# Autodesk Inventor assembly: v2RevA
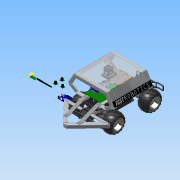
[picture p0: Inventor's stored thumbnail of the model, 180x180]
Saved by Autodesk Inventor 2014 (Build 180170000, 170)
## iProperties
Created: 2013-12-30
Part Number: v2RevA
Document SubType Name: Assembly
Designer: davidgitz
Author: davidgitz
## Documents named in this file (40)
- C:\SharedDrive\Dropbox\ICARUS\Rover\v2-Mechanical\v2RevA.iam
- C:\SharedDrive\Dropbox\ICARUS\Rover\v2-Mechanical\Frame\FrameMember.ipt
- C:\SharedDrive\Dropbox\ICARUS\Rover\v2-Mechanical\Frame\Hex Offset.ipt
- C:\SharedDrive\Dropbox\ICARUS\Rover\v2-Mechanical\Frame\Plate.ipt
- C:\SharedDrive\Dropbox\ICARUS\Rover\v2-Mechanical\Electronics\IFI,VICTOR,Victor 884\IFI,VICTOR,Victor 884.iam
- C:\SharedDrive\Dropbox\ICARUS\Rover\v2-Mechanical\Electronics\FuseBlock.ipt
- C:\SharedDrive\Dropbox\ICARUS\Rover\v2-Mechanical\Electronics\Terminal Block.ipt
- C:\SharedDrive\Dropbox\ICARUS\Rover\v2-Mechanical\H2 OEM\Drive Axle.ipt
- C:\SharedDrive\Dropbox\ICARUS\Rover\v2-Mechanical\H2 OEM\Rear Axle Housing.ipt
- C:\SharedDrive\Dropbox\ICARUS\Rover\v2-Mechanical\H2 OEM\Elec Cover.ipt
- C:\SharedDrive\Dropbox\ICARUS\Rover\v2-Mechanical\H2 OEM\Shock Plate - Top (Left).ipt
- C:\SharedDrive\Dropbox\ICARUS\Rover\v2-Mechanical\H2 OEM\Shock Plate - Bottom (Left).ipt
- C:\SharedDrive\Dropbox\ICARUS\Rover\v2-Mechanical\H2 OEM\Shock Plate - Bottom (Right).ipt
- C:\SharedDrive\Dropbox\ICARUS\Rover\v2-Mechanical\H2 OEM\Shock Plate - Top (Right).ipt
- C:\SharedDrive\Dropbox\ICARUS\Rover\v2-Mechanical\H2 OEM\Shock Mount - Top.ipt
- C:\SharedDrive\Dropbox\ICARUS\Rover\v2-Mechanical\Imported Components\Final\Final.iam
- C:\SharedDrive\Dropbox\ICARUS\Rover\v2-Mechanical\Imported Components\ArduinoMega2560R3\ArduinoMega2560R3.iam
- C:\SharedDrive\Dropbox\ICARUS\Rover\v2-Mechanical\Electronics\GBS-20132-EL2.ipt
- C:\SharedDrive\Dropbox\ICARUS\Rover\v2-Mechanical\H2 OEM\FrontHousing.ipt
- C:\SharedDrive\Dropbox\ICARUS\Rover\v2-Mechanical\H2 OEM\RearHousing.ipt
- C:\SharedDrive\Dropbox\ICARUS\Rover\v2-Mechanical\H2 OEM\LargeLeftWheel.ipt
- C:\SharedDrive\Dropbox\ICARUS\Rover\v2-Mechanical\H2 OEM\LargeRightWheel.ipt
- C:\SharedDrive\Dropbox\ICARUS\Rover\v2-Mechanical\H2 OEM\Front Axle Housing.ipt
- C:\SharedDrive\Dropbox\ICARUS\Rover\v2-Mechanical\H2 OEM\Front Axle Body.ipt
- C:\SharedDrive\Dropbox\ICARUS\Rover\v2-Mechanical\H2 OEM\BackBumper.ipt
- C:\SharedDrive\Dropbox\ICARUS\Rover\v2-Mechanical\H2 OEM\FrontBumper.ipt
- C:\SharedDrive\Dropbox\ICARUS\Rover\v2-Mechanical\H2 OEM\Shock Mount - Bottom.ipt
- C:\SharedDrive\Dropbox\ICARUS\Rover\v2-Mechanical\Frame\FrameBlock.ipt
- C:\SharedDrive\Dropbox\ICARUS\Rover\v2-Mechanical\H2 OEM\Shock Spring.ipt
- C:\SharedDrive\Dropbox\ICARUS\Rover\v2-Mechanical\Frame\FrameMember_MIR.ipt
- C:\SharedDrive\Dropbox\ICARUS\Rover\v2-Mechanical\Frame\FrameBlock_MIR.ipt
- C:\SharedDrive\Dropbox\ICARUS\Rover\v2-Mechanical\Frame\CageFrame.ipt
- C:\SharedDrive\Dropbox\ICARUS\Rover\v2-Mechanical\Frame\SideAccessPanel.ipt
- C:\SharedDrive\Dropbox\ICARUS\Rover\v2-Mechanical\Frame\TopPanel.ipt
- C:\SharedDrive\Dropbox\ICARUS\Rover\v2-Mechanical\Electronics\MainPCB.ipt
- C:\SharedDrive\Dropbox\ICARUS\Rover\v2-Mechanical\Electronics\Maxbotix,LV-MaxSonar-EZ\LV-MaxSonar-EZ.iam
- C:\SharedDrive\Dropbox\ICARUS\Rover\v2-Mechanical\Electronics\3DRobotics,Radio\3DR_Radio_Assy.iam
- C:\SharedDrive\Dropbox\ICARUS\Rover\v2-Mechanical\Frame\Wedge.ipt
- C:\SharedDrive\Dropbox\ICARUS\Rover\v2-Mechanical\Frame\WedgeBrace.ipt
- C:\SharedDrive\Dropbox\ICARUS\Rover\v2-Mechanical\Frame\WedgeBrace_MIR.ipt
## Components (70 placed, 46 different names)
1. Hex Offset:1 — Insert:41
2. Plate:1 — Mate:3, Mate:16, Flush:13, Flush:14, Mate:19, Flush:40, Insert:41, Insert:42, Insert:43, Insert:44, Flush:41, Mate:65, Mate:66, Mate:69, Mate:70, Mate:71
3. IFI,VICTOR,Victor 884:1 [sub-assembly] — Mate:69, Mate:70, Mate:71
4. FuseBlock:1 — Mate:16, Flush:13, Flush:14
5. FrameMember:2 — Mate:61, Flush:36, Flush:37, Mate:63, Flush:38, Flush:39, Mate:64, Flush:42, Flush:56
6. 12V PDB — Mate:19, Flush:41
7. 6V PDB — Mate:66
8. 5V PDB — Mate:65
9. Drive Axle:1 — Mate:9, Insert:2, Insert:36
10. Drive Axle:2 — Mate:7, Insert:1, Insert:35
11. Drive Axle:3 — Mate:13, Insert:6, Insert:25
12. Drive Axle:4 — Mate:11, Insert:5, Insert:26
13. Elec Cover:1 — Flush:43, Mate:67, Mate:68
14. FrontLeft_Wheel — Mate:7, Insert:1
15. FrontRight_Wheel — Mate:9, Insert:2
16. BackLeft_Wheel — Mate:13, Insert:6
17. BackRight_Wheel — Mate:11, Insert:5
18. Shock Plate - Top (Left):1 — Insert:17, Insert:21, Insert:38
19. Shock Plate - Bottom (Left):1 — Insert:18, Insert:22
20. Shock Plate - Bottom (Right):1 — Insert:20, Insert:23
21. Shock Plate - Top (Right):1 — Insert:19, Insert:24, Insert:40
22. Arduino Uno [sub-assembly]
23. ArduinoMega2560R3:1 [sub-assembly] — Mate:78, Flush:52, Flush:54, Flush:55, Mate:79, Flush:57
24. Motor Shield — Flush:54, Flush:55, Mate:79
25. FrontHousing:1 — Insert:13, Insert:15, Angle:4, Flush:16, Insert:27, Insert:28, Mate:22, Flush:17, Mate:23, Mate:25, Angle:5, Flush:18, Flush:19, Mate:29, Mate:31, Flush:31, Flush:58, Flush:59
26. Shock Plate - Bottom (Left):2 — Insert:27, Insert:30
27. Shock Plate - Top (Left):2 — Insert:13, Insert:29, Insert:37
28. Shock Plate - Bottom (Right):2 — Insert:28, Insert:32
29. Shock Plate - Top (Right):2 — Insert:15, Insert:31, Insert:39
30. RearHousing:1 — Insert:17, Insert:18, Insert:19, Insert:20, Mate:22, Flush:17, Mate:23, Mate:24, Flush:20, Mate:27, Mate:34, Mate:35, Mate:61, Flush:36, Mate:67, Mate:68
31. Rear Axle Housing:3 — Insert:21, Insert:22, Insert:25
32. Rear Axle Housing:4 — Insert:23, Insert:24, Insert:26
33. Front Left Axle Housing:1 — Insert:29, Insert:30, Insert:33, DRIVEN-FL WHEEL ANGLE
34. Front Right Axle Housing:2 — Insert:31, Insert:32, Insert:34, DRIVEN-FR WHEEL ANGLE
35. Front Left Axle Body:1 — Insert:33, Insert:35, DRIVEN-FL WHEEL ANGLE
36. Front Right Axle Body:2 — Insert:34, Insert:36, DRIVEN-FR WHEEL ANGLE
37. BackBumper:1 — Flush:20, Mate:27, Flush:21
38. FrontBumper:1 — Mate:26, Angle:5, Flush:18, Flush:19
39. Shock Mount - Bottom:1 — Insert:40, Mate:33, Mate:52
40. Shock Mount - Top:2 — Mate:33, Mate:34, Mate:50, Mate:51
41. Shock Mount - Bottom:2 — Insert:39, Mate:30, Mate:46
42. Shock Mount - Top:3 — Mate:30, Mate:31, Mate:44, Mate:45
43. Shock Mount - Bottom:3 — Insert:37, Mate:28, Mate:41, DRIVEN-SHOCK HEIGHT
44. Shock Mount - Top:4 — Mate:32, Mate:35, Mate:47, Mate:48
45. Shock Mount - Bottom:4 — Insert:38, Mate:32, Mate:49
46. FL Shock Mount — Mate:28, Mate:29, Mate:40, Mate:42, DRIVEN-SHOCK HEIGHT
47. Shock Spring:1 — Mate:40, Mate:41, Mate:42
48. Shock Spring:2 — Mate:44, Mate:45, Mate:46
49. Shock Spring:3 — Mate:47, Mate:48, Mate:49
50. Shock Spring:4 — Mate:50, Mate:51, Mate:52
51. FrameMember_MIR:1 — Mate:62, Flush:40, Flush:42, Flush:44, Mate:72, Mate:77, Flush:56
52. FrameBlock:1 — Mate:63, Flush:38, Flush:39
53. FrameBlock_MIR:1
54. Hex Offset:2 — Insert:42
55. Hex Offset:3 — Insert:43, Mate:64
56. Hex Offset:4 — Insert:44
57. CageFrame:1 — Flush:44, Flush:46, Mate:73, Flush:50
58. CageFrame:2 — Mate:72, Flush:46, Flush:47, Mate:74, Mate:75, Mate:80, Flush:60
59. SideAccessPanel:1 — Flush:47, Flush:49, Mate:75, Mate:80
60. SideAccessPanel:2 — Mate:73, Flush:49, Mate:74
61. TopPanel:1 — Flush:50
62. Hex Offset:5 — Mate:77, Flush:51
63. MainPCB:1 — Flush:51, Mate:78, Flush:52, Flush:57
64. LV-MaxSonar-EZ:1 [sub-assembly]
65. LV-MaxSonar-EZ:2 [sub-assembly]
66. LV-MaxSonar-EZ:3 [sub-assembly]
67. 3DR_Radio_Assy:1 [sub-assembly]
68. Wedge:1 — Flush:59
69. WedgeBrace:1 — Flush:60
70. WedgeBrace_MIR:1
## Relationships (124: Mate 53, Insert 34, Flush 33, Angle 4)
- Flush:5
- Mate:3: Plate:1
- Mate:7: Drive Axle:2 ↔ FrontLeft_Wheel
- Insert:1: Drive Axle:2 ↔ FrontLeft_Wheel
- Mate:9: Drive Axle:1 ↔ FrontRight_Wheel
- Insert:2: Drive Axle:1 ↔ FrontRight_Wheel
- Mate:11: Drive Axle:4 ↔ BackRight_Wheel
- Insert:5: Drive Axle:4 ↔ BackRight_Wheel
- Mate:13: Drive Axle:3 ↔ BackLeft_Wheel
- Insert:6: Drive Axle:3 ↔ BackLeft_Wheel
- Mate:16: Plate:1 ↔ FuseBlock:1
- Flush:13: Plate:1 ↔ FuseBlock:1
- Flush:14: Plate:1 ↔ FuseBlock:1
- Mate:19: Plate:1 ↔ 12V PDB
- Insert:13: FrontHousing:1 ↔ Shock Plate - Top (Left):2
- Insert:15: FrontHousing:1 ↔ Shock Plate - Top (Right):2
- Insert:17: Shock Plate - Top (Left):1 ↔ RearHousing:1
- Insert:18: Shock Plate - Bottom (Left):1 ↔ RearHousing:1
- Insert:19: Shock Plate - Top (Right):1 ↔ RearHousing:1
- Insert:20: Shock Plate - Bottom (Right):1 ↔ RearHousing:1
- Insert:21: Shock Plate - Top (Left):1 ↔ Rear Axle Housing:3
- Insert:22: Shock Plate - Bottom (Left):1 ↔ Rear Axle Housing:3
- Insert:23: Shock Plate - Bottom (Right):1 ↔ Rear Axle Housing:4
- Insert:24: Shock Plate - Top (Right):1 ↔ Rear Axle Housing:4
- Insert:25: Drive Axle:3 ↔ Rear Axle Housing:3
- Insert:26: Drive Axle:4 ↔ Rear Axle Housing:4
- Angle:4 (0 deg): FrontHousing:1
- Flush:16: FrontHousing:1
- Insert:27: FrontHousing:1 ↔ Shock Plate - Bottom (Left):2
- Insert:28: FrontHousing:1 ↔ Shock Plate - Bottom (Right):2
- Insert:29: Shock Plate - Top (Left):2 ↔ Front Left Axle Housing:1
- Insert:30: Shock Plate - Bottom (Left):2 ↔ Front Left Axle Housing:1
- Insert:31: Shock Plate - Top (Right):2 ↔ Front Right Axle Housing:2
- Insert:32: Shock Plate - Bottom (Right):2 ↔ Front Right Axle Housing:2
- Insert:33 (0.6604 mm): Front Left Axle Housing:1 ↔ Front Left Axle Body:1
- Insert:34 (0.6604 mm): Front Right Axle Housing:2 ↔ Front Right Axle Body:2
- Insert:35: Drive Axle:2 ↔ Front Left Axle Body:1
- Insert:36: Drive Axle:1 ↔ Front Right Axle Body:2
- Mate:22: FrontHousing:1 ↔ RearHousing:1
- Flush:17: FrontHousing:1 ↔ RearHousing:1
- Mate:23: FrontHousing:1 ↔ RearHousing:1
- Mate:24: RearHousing:1
- Mate:25: FrontHousing:1
- Mate:26: FrontBumper:1
- Angle:5 (0 deg): FrontHousing:1 ↔ FrontBumper:1
- Flush:18 (2.54 mm): FrontHousing:1 ↔ FrontBumper:1
- Flush:19: FrontHousing:1 ↔ FrontBumper:1
- Flush:20: RearHousing:1 ↔ BackBumper:1
- Mate:27: RearHousing:1 ↔ BackBumper:1
- Flush:21: BackBumper:1
- Insert:37 (0.889 mm): Shock Plate - Top (Left):2 ↔ Shock Mount - Bottom:3
- Insert:38 (0.889 mm): Shock Plate - Top (Left):1 ↔ Shock Mount - Bottom:4
- Insert:39 (0.889 mm): Shock Plate - Top (Right):2 ↔ Shock Mount - Bottom:2
- Insert:40 (0.889 mm): Shock Plate - Top (Right):1 ↔ Shock Mount - Bottom:1
- Mate:28: Shock Mount - Bottom:3 ↔ FL Shock Mount
- Mate:29: FrontHousing:1 ↔ FL Shock Mount
- Mate:30: Shock Mount - Bottom:2 ↔ Shock Mount - Top:3
- Mate:31: FrontHousing:1 ↔ Shock Mount - Top:3
- Mate:32: Shock Mount - Top:4 ↔ Shock Mount - Bottom:4
- Mate:33: Shock Mount - Bottom:1 ↔ Shock Mount - Top:2
- Mate:34: RearHousing:1 ↔ Shock Mount - Top:2
- Mate:35: RearHousing:1 ↔ Shock Mount - Top:4
- Flush:29
- DRIVEN-FL WHEEL ANGLE [Angle] (0 deg): Front Left Axle Housing:1 ↔ Front Left Axle Body:1
- DRIVEN-FR WHEEL ANGLE [Angle] (0 deg): Front Right Axle Housing:2 ↔ Front Right Axle Body:2
- Mate:40: FL Shock Mount ↔ Shock Spring:1
- Mate:41: Shock Mount - Bottom:3 ↔ Shock Spring:1
- Mate:42: FL Shock Mount ↔ Shock Spring:1
- DRIVEN-SHOCK HEIGHT [Mate] (38.1 mm): Shock Mount - Bottom:3 ↔ FL Shock Mount
- Mate:44: Shock Mount - Top:3 ↔ Shock Spring:2
- Mate:45: Shock Mount - Top:3 ↔ Shock Spring:2
- Mate:46: Shock Mount - Bottom:2 ↔ Shock Spring:2
- Mate:47: Shock Mount - Top:4 ↔ Shock Spring:3
- Mate:48: Shock Mount - Top:4 ↔ Shock Spring:3
- Mate:49: Shock Mount - Bottom:4 ↔ Shock Spring:3
- Mate:50: Shock Mount - Top:2 ↔ Shock Spring:4
- Mate:51: Shock Mount - Top:2 ↔ Shock Spring:4
- Mate:52: Shock Mount - Bottom:1 ↔ Shock Spring:4
- Flush:31 (-13.97 mm): FrontHousing:1
- Mate:61: FrameMember:2 ↔ RearHousing:1
- Flush:36 (3.81 mm): FrameMember:2 ↔ RearHousing:1
- Flush:37 (63.5 mm): FrameMember:2
- Mate:62 (-63.5 mm): FrameMember_MIR:1
- Mate:63: FrameMember:2 ↔ FrameBlock:1
- Flush:38: FrameMember:2 ↔ FrameBlock:1
- Flush:39: FrameMember:2 ↔ FrameBlock:1
- Flush:40 (8.382 mm): Plate:1 ↔ FrameMember_MIR:1
- Insert:41: Hex Offset:1 ↔ Plate:1
- Insert:42: Plate:1 ↔ Hex Offset:2
- Insert:43: Plate:1 ↔ Hex Offset:3
- Insert:44: Plate:1 ↔ Hex Offset:4
- Mate:64: FrameMember:2 ↔ Hex Offset:3
- Flush:41: Plate:1 ↔ 12V PDB
- Flush:42: FrameMember:2 ↔ FrameMember_MIR:1
- Mate:65: Plate:1 ↔ 5V PDB
- Mate:66: Plate:1 ↔ 6V PDB
- Flush:43: Elec Cover:1
- Mate:67: Elec Cover:1 ↔ RearHousing:1
- Mate:68: Elec Cover:1 ↔ RearHousing:1
- Mate:69: Plate:1 ↔ IFI,VICTOR,Victor 884:1
- Mate:70 (3.81 mm): Plate:1 ↔ IFI,VICTOR,Victor 884:1
- Mate:71 (6.35 mm): Plate:1 ↔ IFI,VICTOR,Victor 884:1
- Flush:44: FrameMember_MIR:1 ↔ CageFrame:1
- Mate:72: FrameMember_MIR:1 ↔ CageFrame:2
- Flush:46: CageFrame:1 ↔ CageFrame:2
- Flush:47: CageFrame:2 ↔ SideAccessPanel:1
- Mate:73: CageFrame:1 ↔ SideAccessPanel:2
- Flush:49: SideAccessPanel:1 ↔ SideAccessPanel:2
- Mate:74: CageFrame:2 ↔ SideAccessPanel:2
- Mate:75: CageFrame:2 ↔ SideAccessPanel:1
- Flush:50: CageFrame:1 ↔ TopPanel:1
- Mate:77: FrameMember_MIR:1 ↔ Hex Offset:5
- Flush:51: Hex Offset:5 ↔ MainPCB:1
- Mate:78: ArduinoMega2560R3:1 ↔ MainPCB:1
- Flush:52: ArduinoMega2560R3:1 ↔ MainPCB:1
- Flush:54: ArduinoMega2560R3:1 ↔ Motor Shield
- Flush:55: ArduinoMega2560R3:1 ↔ Motor Shield
- Mate:79: ArduinoMega2560R3:1 ↔ Motor Shield
- Flush:56: FrameMember:2 ↔ FrameMember_MIR:1
- Flush:57 (25.4 mm): ArduinoMega2560R3:1 ↔ MainPCB:1
- Flush:58: FrontHousing:1
- Flush:59: FrontHousing:1 ↔ Wedge:1
- Mate:80: CageFrame:2 ↔ SideAccessPanel:1
- Flush:60: CageFrame:2 ↔ WedgeBrace:1
